# Autodesk Inventor assembly: Drumstick
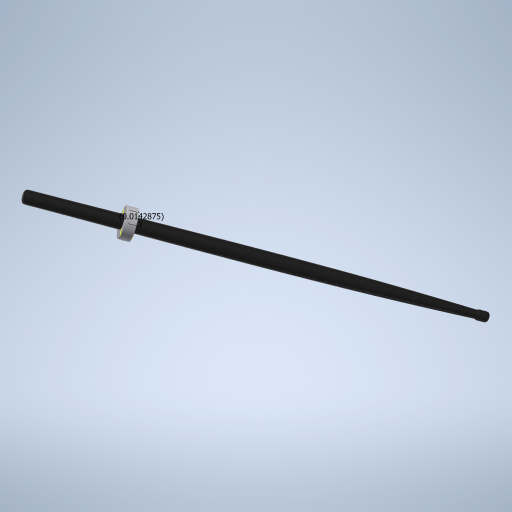
[picture p0: Inventor's stored thumbnail of the model, 512x512]
Saved by Autodesk Inventor 2023 (Build 270158000, 158)
## iProperties
Created: 2020-03-24
Part Number: Drumstick
Document SubType Name: Assembly
Designer: valer
Mass: 71.6665 g
Surface Area: 198.912 cm^2
Volume: 58.3702 cm^3
Density: 1.22779 g/cm^3
Author: valer
## Documents named in this file (4)
- C:\Users\LattePanda\Desktop\str1ker\cad\Drumstick.iam
- C:\Users\LattePanda\Desktop\str1ker\cad\external\Drumstick\Drumstick.ipt
- C:\Users\LattePanda\Desktop\str1ker\cad\external\ForearmShaftCollar.ipt
- C:\Users\LattePanda\Desktop\str1ker\cad\external\Drumstick\DrumstickBoundingBox.ipt
## Components (3 placed, 3 different names)
1. Drumstick:1 — Flush:3, Mate:84, Angle:1, Angle:2, Mate:85, Mate:87
2. ShaftCollar1/2:1 — Flush:3, Mate:84, Angle:3, Mate:86, Flush:4
3. DrumstickBoundingBox:1 — Mate:87, Flush:4
## Relationships (9: Mate 4, Angle 3, Flush 2)
- Flush:3 (304.8 mm): Drumstick:1 ↔ ShaftCollar1/2:1
- Mate:84: Drumstick:1 ↔ ShaftCollar1/2:1
- Angle:1 (180 deg): Drumstick:1
- Angle:2 (180 deg): Drumstick:1
- Mate:85: Drumstick:1
- Angle:3 (180 deg): ShaftCollar1/2:1
- Mate:86: ShaftCollar1/2:1
- Mate:87: Drumstick:1 ↔ DrumstickBoundingBox:1
- Flush:4: ShaftCollar1/2:1 ↔ DrumstickBoundingBox:1
